# Autodesk Inventor assembly: JH_Greifer_Scheibe_final
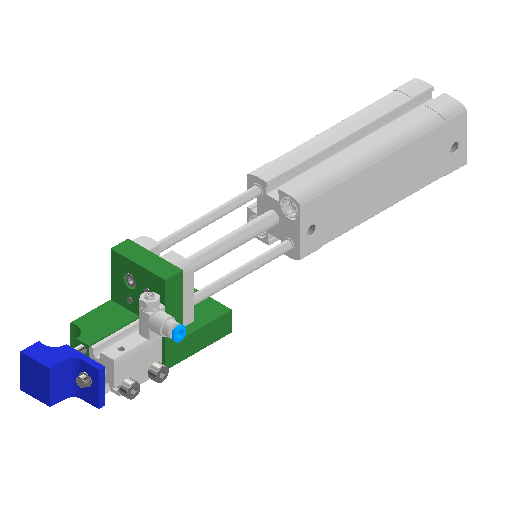
[picture p0: Inventor's stored thumbnail of the model, 512x512]
Saved by Autodesk Inventor 2025.1 (Build 291241000, 241)
## iProperties
Created: 2025-06-22
Part Number: JH_Greifer_Scheibe_final
Document SubType Name: Assembly
Designer: Jakob
Author: Jakob
## Documents named in this file (12)
- C:\Users\Erik\Erik\Hochschule\3. Semester\CAD\CAD-Paspa\Useless Box\Eigene Bauteile\JH_Greifer_Unterlegscheibe\Eigene Bauteile\JH_Greifer_Scheibe_final.iam
- C:\Users\Erik\Erik\Hochschule\3. Semester\CAD\CAD-Paspa\Useless Box\Eigene Bauteile\JH_Greifer_Unterlegscheibe\Eigene Bauteile\JH_int_Adapterplatte.ipt
- C:\Users\Erik\Erik\Hochschule\3. Semester\CAD\CAD-Paspa\Useless Box\Standart Bauteile\DIN EN ISO 4762 - M3 x 10.ipt
- C:\Users\Erik\Erik\Hochschule\3. Semester\CAD\CAD-Paspa\Useless Box\Standart Bauteile\DIN EN ISO 2338 - 3 h8 x 14.ipt
- C:\Users\Erik\Erik\Hochschule\3. Semester\CAD\CAD-Paspa\Useless Box\Standart Bauteile\DIN EN ISO 2338 - 4 h8 x 14.ipt
- C:\Users\Erik\Erik\Hochschule\3. Semester\CAD\CAD-Paspa\Useless Box\Eigene Bauteile\JH_Greifer_Unterlegscheibe\Eigene Bauteile\JH_int_Greiferkoerper_Gegenstueck.ipt
- C:\Users\Erik\Erik\Hochschule\3. Semester\CAD\CAD-Paspa\Useless Box\Eigene Bauteile\JH_Greifer_Unterlegscheibe\Kaufteile\AIS2024\5267300 AEN-S-6-5-I-A---(0_high).iam
- C:\Users\Erik\Erik\Hochschule\3. Semester\CAD\CAD-Paspa\Useless Box\Standart Bauteile\DIN EN ISO 4762 - M2,5 x 5.ipt
- C:\Users\Erik\Erik\Hochschule\3. Semester\CAD\CAD-Paspa\Useless Box\Standart Bauteile\DIN 125 - A 2,7.ipt
- C:\Users\Erik\Erik\Hochschule\3. Semester\CAD\CAD-Paspa\Useless Box\Standart Bauteile\DIN EN ISO 4762 - M4 x 16.ipt
- C:\Users\Erik\Erik\Hochschule\3. Semester\CAD\CAD-Paspa\Useless Box\Eigene Bauteile\JH_Greifer_Unterlegscheibe\Kaufteile\Drosselrückschlagventil\175043 GRLZ-M3-QS-3.ipt
- C:\Users\Erik\Erik\Hochschule\3. Semester\CAD\CAD-Paspa\Useless Box\Eigene Bauteile\JH_Greifer_Unterlegscheibe\Kaufteile\Führungszylinder\Zylinder_50mm\AIS2024\537123 ADNGF-12-50-P-A---(0)_50mm.iam
## Components (15 placed, 11 different names)
1. JH_int_Adapterplatte:1 — Passend:6, Passend:7, Passend:8, Passend:9, Passend:10, Passend:11, Fluchtend:2, Fluchtend:3, Passend:12, Passend:13, Passend:14, Passend:15, Passend:18, Passend:19, Passend:20, Passend:33, Passend:34, Passend:35
2. DIN EN ISO 4762 - M3 x 10:1 — Passend:6, Passend:7
3. DIN EN ISO 4762 - M3 x 10:2 — Passend:8, Passend:9
4. DIN EN ISO 2338 - 3 h8 x 14:1 — Passend:10, Fluchtend:2
5. DIN EN ISO 2338 - 3 h8 x 14:2 — Passend:11, Fluchtend:3
6. DIN EN ISO 2338 - 4 h8 x 14:1 — Passend:12, Passend:14, Passend:16
7. DIN EN ISO 2338 - 4 h8 x 14:2 — Passend:13, Passend:15, Passend:17
8. JH_int_Greiferkoerper_Gegenstueck:1 — Passend:16, Passend:17, Fluchtend:4, Passend:21
9. 5267300 AEN-S-6-5-I-A---(0_high):1 [sub-assembly] — Passend:18, Passend:19, Passend:20, Fluchtend:4, Passend:22, Passend:23, Passend:25, Passend:26, Passend:27, Passend:28, Passend:29, Passend:30
10. DIN EN ISO 4762 - M2,5 x 5:1 — Passend:23, Passend:24
11. DIN 125 - A 2,7:1 — Passend:21, Passend:22, Passend:24
12. DIN EN ISO 4762 - M4 x 16:1 — Passend:25, Passend:27
13. DIN EN ISO 4762 - M4 x 16:2 — Passend:26, Passend:28
14. 175043 GRLZ-M3-QS-3:1 — Passend:29, Passend:30, Winkel:1
15. 537123 ADNGF-12-50-P-A---(0)_50mm:1 [sub-assembly] — Passend:31, Passend:32, Fluchtend:7, Passend:33, Passend:34, Passend:35
## Relationships (35: Mate 30, Flush 4, Angle 1)
- Passend:6 [Mate]: JH_int_Adapterplatte:1 ↔ DIN EN ISO 4762 - M3 x 10:1
- Passend:7 [Mate]: JH_int_Adapterplatte:1 ↔ DIN EN ISO 4762 - M3 x 10:1
- Passend:8 [Mate]: JH_int_Adapterplatte:1 ↔ DIN EN ISO 4762 - M3 x 10:2
- Passend:9 [Mate]: JH_int_Adapterplatte:1 ↔ DIN EN ISO 4762 - M3 x 10:2
- Passend:10 [Mate]: JH_int_Adapterplatte:1 ↔ DIN EN ISO 2338 - 3 h8 x 14:1
- Passend:11 [Mate]: JH_int_Adapterplatte:1 ↔ DIN EN ISO 2338 - 3 h8 x 14:2
- Fluchtend:2 [Flush]: JH_int_Adapterplatte:1 ↔ DIN EN ISO 2338 - 3 h8 x 14:1
- Fluchtend:3 [Flush]: JH_int_Adapterplatte:1 ↔ DIN EN ISO 2338 - 3 h8 x 14:2
- Passend:12 [Mate]: JH_int_Adapterplatte:1 ↔ DIN EN ISO 2338 - 4 h8 x 14:1
- Passend:13 [Mate]: JH_int_Adapterplatte:1 ↔ DIN EN ISO 2338 - 4 h8 x 14:2
- Passend:14 [Mate]: JH_int_Adapterplatte:1 ↔ DIN EN ISO 2338 - 4 h8 x 14:1
- Passend:15 [Mate]: JH_int_Adapterplatte:1 ↔ DIN EN ISO 2338 - 4 h8 x 14:2
- Passend:16 [Mate]: DIN EN ISO 2338 - 4 h8 x 14:1 ↔ JH_int_Greiferkoerper_Gegenstueck:1
- Passend:17 [Mate]: DIN EN ISO 2338 - 4 h8 x 14:2 ↔ JH_int_Greiferkoerper_Gegenstueck:1
- Passend:18 [Mate]: JH_int_Adapterplatte:1 ↔ 5267300 AEN-S-6-5-I-A---(0_high):1
- Passend:19 [Mate]: JH_int_Adapterplatte:1 ↔ 5267300 AEN-S-6-5-I-A---(0_high):1
- Passend:20 [Mate]: JH_int_Adapterplatte:1 ↔ 5267300 AEN-S-6-5-I-A---(0_high):1
- Fluchtend:4 [Flush]: JH_int_Greiferkoerper_Gegenstueck:1 ↔ 5267300 AEN-S-6-5-I-A---(0_high):1
- Passend:21 [Mate]: JH_int_Greiferkoerper_Gegenstueck:1 ↔ DIN 125 - A 2,7:1
- Passend:22 [Mate]: 5267300 AEN-S-6-5-I-A---(0_high):1 ↔ DIN 125 - A 2,7:1
- Passend:23 [Mate]: 5267300 AEN-S-6-5-I-A---(0_high):1 ↔ DIN EN ISO 4762 - M2,5 x 5:1
- Passend:24 [Mate]: DIN EN ISO 4762 - M2,5 x 5:1 ↔ DIN 125 - A 2,7:1
- Passend:25 [Mate]: 5267300 AEN-S-6-5-I-A---(0_high):1 ↔ DIN EN ISO 4762 - M4 x 16:1
- Passend:26 [Mate]: 5267300 AEN-S-6-5-I-A---(0_high):1 ↔ DIN EN ISO 4762 - M4 x 16:2
- Passend:27 [Mate]: 5267300 AEN-S-6-5-I-A---(0_high):1 ↔ DIN EN ISO 4762 - M4 x 16:1
- Passend:28 [Mate]: 5267300 AEN-S-6-5-I-A---(0_high):1 ↔ DIN EN ISO 4762 - M4 x 16:2
- Passend:29 [Mate]: 5267300 AEN-S-6-5-I-A---(0_high):1 ↔ 175043 GRLZ-M3-QS-3:1
- Passend:30 [Mate]: 5267300 AEN-S-6-5-I-A---(0_high):1 ↔ 175043 GRLZ-M3-QS-3:1
- Winkel:1 [Angle] (0 deg): 175043 GRLZ-M3-QS-3:1
- Passend:31 [Mate]: 537123 ADNGF-12-50-P-A---(0)_50mm:1
- Passend:32 [Mate]: 537123 ADNGF-12-50-P-A---(0)_50mm:1
- Fluchtend:7 [Flush]: 537123 ADNGF-12-50-P-A---(0)_50mm:1
- Passend:33 [Mate]: JH_int_Adapterplatte:1 ↔ 537123 ADNGF-12-50-P-A---(0)_50mm:1
- Passend:34 [Mate]: JH_int_Adapterplatte:1 ↔ 537123 ADNGF-12-50-P-A---(0)_50mm:1
- Passend:35 [Mate]: JH_int_Adapterplatte:1 ↔ 537123 ADNGF-12-50-P-A---(0)_50mm:1
